# Autodesk Inventor assembly: Body 2.0
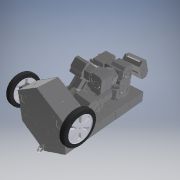
[picture p0: Inventor's stored thumbnail of the model, 180x180]
Saved by Autodesk Inventor 2017 (Build 210142000, 142)
## iProperties
Created: 2019-05-22
Part Number: Body 2.0
Document SubType Name: Assembly
Designer: Dell
Mass: 18970.5 g
Surface Area: 54771 cm^2
Volume: 19738.1 cm^3
Density: 0.961113 g/cm^3
Author: Dell
## Documents named in this file (43)
- C:\Users\Dell\Documents\GitHub\tr2\Body 2.0\Body 2.0.iam
- C:\Users\Dell\Documents\GitHub\tr2\Body 2.0\BA01.ipt
- C:\Users\Dell\Documents\GitHub\tr2\Body 2.0\BA02.ipt
- C:\Users\Dell\Documents\GitHub\tr2\Body 2.0\BA03.ipt
- C:\Users\Dell\Documents\GitHub\tr2\Body 2.0\BA04.ipt
- C:\Users\Dell\Documents\GitHub\tr2\Body 2.0\BA05.ipt
- C:\Users\Dell\Documents\GitHub\tr2\Body 2.0\BA06.ipt
- C:\Users\Dell\Documents\GitHub\tr2\Body 2.0\BA07.ipt
- C:\Users\Dell\Documents\GitHub\tr2\Body 2.0\BA08.ipt
- C:\Users\Dell\Documents\GitHub\tr2\Body 2.0\ST01.ipt
- C:\Users\Dell\Documents\GitHub\tr2\Actuator 1.3\Actuator 1.3.iam
- C:\Users\Dell\Documents\GitHub\tr2\Body 2.0\AE01.ipt
- C:\Users\Dell\Documents\GitHub\tr2\Body 2.0\BA09.ipt
- C:\Users\Dell\Documents\GitHub\tr2\Body 2.0\BA10.ipt
- C:\Users\Dell\Documents\GitHub\tr2\Body 2.0\BA11.ipt
- C:\Users\Dell\Documents\GitHub\tr2\Body 2.0\BA12.ipt
- C:\Users\Dell\Documents\GitHub\tr2\Body 2.0\BA13.ipt
- C:\Users\Dell\Documents\GitHub\tr2\Body 2.0\BA14.ipt
- C:\Users\Dell\Documents\GitHub\tr2\Body 2.0\BA15.ipt
- C:\Users\Dell\Documents\GitHub\tr2\Body 2.0\BA16.ipt
- C:\Users\Dell\Documents\GitHub\tr2\Body 2.0\BA18.ipt
- C:\Users\Dell\Documents\GitHub\tr2\Body 2.0\BA20.ipt
- C:\Users\Dell\Documents\GitHub\tr2\Body 2.0\BA19.ipt
- C:\Users\Dell\Documents\GitHub\tr2\Body 2.0\BA21.ipt
- C:\Users\Dell\Documents\GitHub\tr2\Body 2.0\Battery_278Wh.ipt
- C:\Users\Dell\Documents\GitHub\tr2\Body 2.0\NVIDIA Jetson TX2.ipt
- C:\Users\Dell\Documents\GitHub\tr2\Body 2.0\BA22.ipt
- C:\Users\Dell\Documents\GitHub\tr2\Wheel Assembly\Wheel Assembly, Left.iam
- C:\Users\Dell\Documents\GitHub\tr2\Wheel Assembly\Wheel Assembly, Right.iam
- C:\Users\Dell\Documents\GitHub\tr2\Base\Caster Wheel\004. Castor Wheel Full_TOP.iam
- C:\Users\Dell\Documents\GitHub\tr2\Head\Head.iam
- C:\Users\Dell\Documents\GitHub\tr2\Arm\Arm.iam
- C:\Users\Dell\Documents\GitHub\tr2\Base\BA27.ipt
- C:\Users\Dell\Documents\GitHub\tr2\Base\HDMI Port.ipt
- C:\Users\Dell\slaterobots.com\Slate Robotics OneDrive - Documents\Autodesk Inventor\tr2-rs1\Base\Power Switch\Power Switch.iam
- C:\Users\Dell\Documents\GitHub\tr2\Body 2.0\BA17b.ipt
- C:\Users\Dell\Documents\GitHub\tr2\Body 2.0\BA23.ipt
- C:\Users\Dell\Documents\GitHub\tr2\Body 2.0\BA28.ipt
- C:\Users\Dell\Documents\GitHub\tr2\Body 2.0\BA29.ipt
- C:\Users\Dell\Documents\GitHub\tr2\Arm 1.1\Arm 1.1.iam
- C:\Users\Dell\Documents\GitHub\tr2\Body 2.0\BA30.ipt
- C:\Users\Dell\Documents\GitHub\tr2\Actuator 2.0\XT-LG.iam
- C:\Users\Dell\Documents\GitHub\tr2\Body 2.0\12 in Wheel.ipt
## Components (52 placed, 42 different names)
1. BA01:1 — Mate:1, Flush:1, Flush:2, Mate:2, Flush:3, Flush:4, Mate:4, Mate:10, Flush:11, Mate:52
2. BA02:1 — Mate:1, Flush:1, Flush:2, Mate:3, Mate:9, Mate:13, Mate:14, Mate:36, Mate:37, Mate:38, Flush:13, Mate:95, Mate:96, Mate:97
3. BA03:1 — Mate:2, Mate:3, Flush:3, Mate:5, Mate:15, Mate:31, Angle:1, Flush:47
4. BA04:1 — Flush:4, Mate:4, Mate:5, Mate:7, Mate:32, Mate:39, Mate:40, Mate:41, Flush:19, Flush:26, Flush:46, Mate:131, Mate:132, Mate:133
5. BA05:1 — Mate:7, Mate:33, Mate:34, Mate:35, Mate:52, Flush:44
6. BA06:1 — Mate:9, Mate:10, Mate:12, Flush:11, Flush:14, Flush:45
7. BA07:1 — Mate:12, Mate:13, Mate:26, Mate:27, Flush:9, Flush:10, Mate:28, Mate:29, Mate:30, Flush:26, Mate:98, Mate:134
8. BA08:1 — Mate:14, Mate:15, Mate:21, Mate:23, Mate:24, Mate:25, Mate:31
9. ST01:1 — Mate:32, Mate:39, Mate:40, Mate:41
10. ST01:2 — Mate:33, Mate:34, Mate:35
11. ST01:3 — Mate:21, Mate:36, Mate:37, Mate:38
12. ST01:4 — Mate:77, Mate:78, Flush:36, Mate:124
13. ST01:5 — Flush:37, Mate:79, Mate:80
14. ST01:6 — Mate:81, Mate:82, Flush:38, Mate:123
15. Actuator 1.3:1 [sub-assembly] — Mate:23, Mate:24, Mate:25, Mate:93, Mate:94
16. AE01:1 — Mate:27, Flush:9, Mate:29
17. AE01:2 — Mate:26, Flush:10, Mate:28, Mate:30
18. BA09:1 — Flush:13, Mate:42, Mate:46, Flush:22, Mate:51, Mate:53, Mate:58, Flush:32, Mate:64, Mate:66, Mate:71, Mate:107, Mate:108, Flush:42, Mate:115, Mate:119, Mate:123, Mate:138, Mate:142
19. BA10:1 — Flush:14, Mate:42, Flush:18, Flush:25, Mate:59, Mate:67, Flush:39, Mate:118, Mate:122, Flush:45, Mate:128, Flush:51
20. BA11:1 — Flush:18, Flush:20, Flush:35, Mate:76, Mate:78, Mate:104, Mate:105, Mate:106, Mate:124, Flush:44, Mate:128, Mate:129, Mate:135, Mate:136, Mate:137
21. BA12:1 — Flush:19, Flush:20, Mate:74, Mate:75, Mate:79, Flush:46, Mate:129
22. BA13:1 — Mate:46, Flush:22, Flush:24, Mate:50, Mate:54, Flush:27, Flush:34, Mate:65, Flush:40, Mate:114, Mate:116, Flush:47, Mate:127, Flush:49, Flush:50
23. BA14:2 — Flush:24, Mate:62, Flush:48, Mate:126, Mate:127
24. BA15:1 — Mate:50, Flush:25, Mate:51, Mate:84, Mate:85, Mate:113, Mate:122, Flush:43, Flush:48
25. BA16:1 — Mate:53, Mate:54, Flush:27, Flush:30, Mate:83
26. BA18:1 — Flush:30, Mate:58, Mate:59, Flush:32
27. BA17b:1 — Mate:113, Mate:125, Flush:43, Mate:126, Mate:147
28. BA20:1 — Flush:34, Mate:62, Mate:68, Mate:70, Mate:86, Mate:87, Mate:90, Mate:91, Mate:92, Mate:99, Mate:125, Mate:130, Mate:143, Mate:145
29. BA19:1 — Mate:64, Flush:35, Mate:65, Mate:77, Flush:36, Flush:37, Mate:80, Mate:81, Mate:82, Flush:38, Mate:98, Mate:109, Mate:134
30. BA19:2 — Mate:74, Mate:75, Mate:76
31. BA21:1 — Mate:66, Mate:67, Mate:71, Mate:72, Mate:73
32. BA22:1 — Mate:83, Mate:84, Mate:85
33. BA23:1 — Mate:114, Mate:115, Mate:116, Mate:117
34. BA23:2 — Mate:118, Mate:119
35. BA27:1 — Mate:104, Mate:105, Mate:106
36. Battery_278Wh:1 — Mate:68, Mate:72, Mate:73
37. NVIDIA Jetson TX2:1 — Mate:70, Mate:107, Mate:108
38. Wheel Assembly, Left:1 [sub-assembly] — Mate:86, Flush:39, Mate:130
39. Wheel Assembly, Right:1 [sub-assembly] — Mate:87, Flush:40, Mate:117
40. 004. Castor Wheel Full_TOP:1 [sub-assembly] — Mate:90, Mate:91, Mate:92
41. Head:1 [sub-assembly] — Mate:93, Mate:94, Angle:1
42. Arm:1 [sub-assembly] — Mate:95, Mate:96, Mate:97
43. HDMI Port:1
44. Power Switch:1 [sub-assembly]
45. BA28:1 — Mate:131, Mate:132, Mate:133
46. BA29:1 — Mate:135, Mate:136, Mate:137
47. Arm 1.1:1 [sub-assembly] — Mate:140, Mate:141
48. BA30:1 — Mate:138, Flush:49, Mate:140, Mate:141, Mate:142
49. XT-LG:1 [sub-assembly] — Flush:50, Mate:143, Mate:144, Mate:146
50. 12 in Wheel:1 — Mate:144
51. XT-LG:2 [sub-assembly] — Mate:145, Mate:146, Flush:51, Mate:147, Mate:148
52. 12 in Wheel:2 — Mate:148
## Relationships (157: Mate 118, Flush 37, Angle 2)
- Mate:1: BA01:1 ↔ BA02:1
- Flush:1: BA01:1 ↔ BA02:1
- Flush:2: BA01:1 ↔ BA02:1
- Mate:2: BA01:1 ↔ BA03:1
- Mate:3: BA02:1 ↔ BA03:1
- Flush:3: BA01:1 ↔ BA03:1
- Flush:4: BA01:1 ↔ BA04:1
- Mate:4: BA01:1 ↔ BA04:1
- Mate:5: BA03:1 ↔ BA04:1
- Mate:7: BA04:1 ↔ BA05:1
- Mate:9: BA02:1 ↔ BA06:1
- Mate:10: BA01:1 ↔ BA06:1
- Mate:12 (1.27 mm): BA06:1 ↔ BA07:1
- Mate:13 (1.27 mm): BA02:1 ↔ BA07:1
- Mate:14 (1.27 mm): BA02:1 ↔ BA08:1
- Mate:15 (1.27 mm): BA03:1 ↔ BA08:1
- Mate:21: BA08:1 ↔ ST01:3
- Mate:23: BA08:1 ↔ Actuator 1.3:1
- Mate:24: BA08:1 ↔ Actuator 1.3:1
- Mate:25: BA08:1 ↔ Actuator 1.3:1
- Mate:26: BA07:1 ↔ AE01:2
- Mate:27: BA07:1 ↔ AE01:1
- Flush:9: BA07:1 ↔ AE01:1
- Flush:10: BA07:1 ↔ AE01:2
- Mate:28: BA07:1 ↔ AE01:2
- Mate:29: BA07:1 ↔ AE01:1
- Mate:30: BA07:1 ↔ AE01:2
- Flush:11: BA01:1 ↔ BA06:1
- Mate:31 (1.27 mm): BA03:1 ↔ BA08:1
- Mate:32: BA04:1 ↔ ST01:1
- Mate:33: BA05:1 ↔ ST01:2
- Mate:34: BA05:1 ↔ ST01:2
- Mate:35: BA05:1 ↔ ST01:2
- Mate:36: BA02:1 ↔ ST01:3
- Mate:37: BA02:1 ↔ ST01:3
- Mate:38: BA02:1 ↔ ST01:3
- Mate:39: BA04:1 ↔ ST01:1
- Mate:40: BA04:1 ↔ ST01:1
- Mate:41: BA04:1 ↔ ST01:1
- Flush:13: BA02:1 ↔ BA09:1
- Flush:14: BA06:1 ↔ BA10:1
- Mate:42: BA09:1 ↔ BA10:1
- Flush:18: BA10:1 ↔ BA11:1
- Flush:19: BA04:1 ↔ BA12:1
- Flush:20: BA11:1 ↔ BA12:1
- Mate:46: BA09:1 ↔ BA13:1
- Flush:22: BA09:1 ↔ BA13:1
- Flush:24: BA13:1 ↔ BA14:2
- Mate:50: BA13:1 ↔ BA15:1
- Flush:25: BA10:1 ↔ BA15:1
- Mate:51: BA09:1 ↔ BA15:1
- Mate:52: BA01:1 ↔ BA05:1
- Flush:26: BA04:1 ↔ BA07:1
- Mate:53: BA09:1 ↔ BA16:1
- Mate:54 (95.25 mm): BA13:1 ↔ BA16:1
- Flush:27: BA13:1 ↔ BA16:1
- Flush:30: BA16:1 ↔ BA18:1
- Mate:58: BA09:1 ↔ BA18:1
- Mate:59 (95.25 mm): BA10:1 ↔ BA18:1
- Flush:32: BA09:1 ↔ BA18:1
- Flush:34: BA13:1 ↔ BA20:1
- Mate:62: BA14:2 ↔ BA20:1
- Mate:64: BA09:1 ↔ BA19:1
- Flush:35: BA11:1 ↔ BA19:1
- Mate:65: BA13:1 ↔ BA19:1
- Mate:66: BA09:1 ↔ BA21:1
- Mate:67: BA10:1 ↔ BA21:1
- Mate:68: BA20:1 ↔ Battery_278Wh:1
- Mate:70: BA20:1 ↔ NVIDIA Jetson TX2:1
- Mate:71 (1.27 mm): BA09:1 ↔ BA21:1
- Mate:72: BA21:1 ↔ Battery_278Wh:1
- Mate:73 (2.5 mm): BA21:1 ↔ Battery_278Wh:1
- Mate:74 (1.27 mm): BA12:1 ↔ BA19:2
- Mate:75: BA12:1 ↔ BA19:2
- Mate:76: BA11:1 ↔ BA19:2
- Mate:77 (1.27 mm): ST01:4 ↔ BA19:1
- Mate:78: ST01:4 ↔ BA11:1
- Flush:36: ST01:4 ↔ BA19:1
- Flush:37: ST01:5 ↔ BA19:1
- Mate:79: ST01:5 ↔ BA12:1
- Mate:80 (1.27 mm): ST01:5 ↔ BA19:1
- Mate:81: ST01:6 ↔ BA19:1
- Mate:82 (1.27 mm): ST01:6 ↔ BA19:1
- Flush:38: ST01:6 ↔ BA19:1
- Mate:83: BA16:1 ↔ BA22:1
- Mate:84 (3.175 mm): BA15:1 ↔ BA22:1
- Mate:85 (3.175 mm): BA15:1 ↔ BA22:1
- Mate:86: BA20:1 ↔ Wheel Assembly, Left:1
- Flush:39: BA10:1 ↔ Wheel Assembly, Left:1
- Mate:87: BA20:1 ↔ Wheel Assembly, Right:1
- Flush:40: BA13:1 ↔ Wheel Assembly, Right:1
- Mate:90: BA20:1 ↔ 004. Castor Wheel Full_TOP:1
- Mate:91: BA20:1 ↔ 004. Castor Wheel Full_TOP:1
- Mate:92: BA20:1 ↔ 004. Castor Wheel Full_TOP:1
- Mate:93: Actuator 1.3:1 ↔ Head:1
- Mate:94: Actuator 1.3:1 ↔ Head:1
- Angle:1 (0 deg): BA03:1 ↔ Head:1
- Mate:95: BA02:1 ↔ Arm:1
- Mate:96: BA02:1 ↔ Arm:1
- Mate:97: BA02:1 ↔ Arm:1
- Mate:98: BA07:1 ↔ BA19:1
- Mate:99: BA20:1
- [Mate]: BA27:1 ↔ Power Switch:1
- [Mate]: BA27:1 ↔ Power Switch:1
- [Angle] (0 deg): BA27:1 ↔ Power Switch:1
- [Mate] (1 mm): BA27:1 ↔ HDMI Port:1
- [Mate] (1 mm): BA27:1 ↔ HDMI Port:1
- [Flush]: BA27:1 ↔ HDMI Port:1
- Mate:104: BA11:1 ↔ BA27:1
- Mate:105: BA11:1 ↔ BA27:1
- Mate:106: BA11:1 ↔ BA27:1
- Mate:107: BA09:1 ↔ NVIDIA Jetson TX2:1
- Mate:108: BA09:1 ↔ NVIDIA Jetson TX2:1
- Flush:42: BA09:1
- Mate:109: BA19:1
- Mate:113: BA15:1 ↔ BA17b:1
- Mate:114 (1.27 mm): BA13:1 ↔ BA23:1
- Mate:115: BA09:1 ↔ BA23:1
- Mate:116: BA13:1 ↔ BA23:1
- Mate:117: BA23:1 ↔ Wheel Assembly, Right:1
- Mate:118 (1.27 mm): BA10:1 ↔ BA23:2
- Mate:119: BA09:1 ↔ BA23:2
- Mate:122: BA10:1 ↔ BA15:1
- Mate:123: ST01:6 ↔ BA09:1
- Mate:124: ST01:4 ↔ BA11:1
- Mate:125: BA17b:1 ↔ BA20:1
- Flush:43: BA15:1 ↔ BA17b:1
- Flush:44: BA05:1 ↔ BA11:1
- Flush:45: BA06:1 ↔ BA10:1
- Flush:46: BA04:1 ↔ BA12:1
- Flush:47: BA03:1 ↔ BA13:1
- Flush:48: BA14:2 ↔ BA15:1
- Mate:126 (1.27 mm): BA14:2 ↔ BA17b:1
- Mate:127 (1.27 mm): BA13:1 ↔ BA14:2
- Mate:128 (1.27 mm): BA10:1 ↔ BA11:1
- Mate:129 (1.27 mm): BA11:1 ↔ BA12:1
- Mate:130: BA20:1 ↔ Wheel Assembly, Left:1
- Mate:131 (1 mm): BA04:1 ↔ BA28:1
- Mate:132 (1 mm): BA04:1 ↔ BA28:1
- Mate:133: BA04:1 ↔ BA28:1
- Mate:134: BA07:1 ↔ BA19:1
- Mate:135 (1 mm): BA11:1 ↔ BA29:1
- Mate:136 (1 mm): BA11:1 ↔ BA29:1
- Mate:137: BA11:1 ↔ BA29:1
- Mate:138: BA09:1 ↔ BA30:1
- Flush:49 (100 mm): BA13:1 ↔ BA30:1
- Mate:140: Arm 1.1:1 ↔ BA30:1
- Mate:141: Arm 1.1:1 ↔ BA30:1
- Mate:142: BA09:1 ↔ BA30:1
- Flush:50: BA13:1 ↔ XT-LG:1
- Mate:143: BA20:1 ↔ XT-LG:1
- Mate:144: XT-LG:1 ↔ 12 in Wheel:1
- Mate:145: BA20:1 ↔ XT-LG:2
- Mate:146: XT-LG:1 ↔ XT-LG:2
- Flush:51: BA10:1 ↔ XT-LG:2
- Mate:147: BA17b:1 ↔ XT-LG:2
- Mate:148: XT-LG:2 ↔ 12 in Wheel:2
## Named parameters: Panel_Thickness = 6.35 mm, Fit_Tolerance = 1.27 mm, Tool_Dia = 6.35 mm, iTrigger0 = 1
